# Autodesk Inventor assembly: Wechselmechnanik
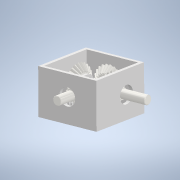
[picture p0: Inventor's stored thumbnail of the model, 180x180]
Saved by Autodesk Inventor 2021 (Build 250183000, 183)
## iProperties
Created: 2021-01-24
Part Number: Wechselmechnanik
Document SubType Name: Assembly
Designer: Jaro Machnow
Author: Jaro Machnow
## Documents named in this file (14)
- C:\Users\LETPJG\Documents\Inventor\zahnstange\Amphibienfahrzeug\Wechsel zwischen Land und Wasser\Mechanik_zum_Wechseln\Wechselmechnanik\Wechselmechnanik.iam
- C:\Users\LETPJG\Documents\Inventor\zahnstange\Amphibienfahrzeug\Wechsel zwischen Land und Wasser\Mechanik_zum_Wechseln\Wechselmechnanik\Konstruktions-Assistent\Kegelräder1.iam
- C:\Users\LETPJG\Documents\Inventor\zahnstange\Amphibienfahrzeug\Wechsel zwischen Land und Wasser\Mechanik_zum_Wechseln\Welle1.ipt
- C:\Users\LETPJG\Documents\Inventor\zahnstange\Amphibienfahrzeug\Wechsel zwischen Land und Wasser\Mechanik_zum_Wechseln\Welle2.ipt
- C:\Users\LETPJG\Documents\Inventor\zahnstange\Amphibienfahrzeug\Wechsel zwischen Land und Wasser\Mechanik_zum_Wechseln\Wechselmechnanik\Konstruktions-Assistent\Lager1.iam
- C:\Users\LETPJG\Documents\Inventor\zahnstange\Amphibienfahrzeug\Wechsel zwischen Land und Wasser\Mechanik_zum_Wechseln\Wechselmechnanik\Konstruktions-Assistent\Kegelräder3.iam
- C:\Users\LETPJG\Documents\Inventor\zahnstange\Amphibienfahrzeug\Wechsel zwischen Land und Wasser\Wechselmechanik\Klappmechanismus\Lager1.iam
- C:\Users\LETPJG\Documents\Inventor\zahnstange\Amphibienfahrzeug\Wechsel zwischen Land und Wasser\Mechanik_zum_Wechseln\Hülle.ipt
- C:\Users\LETPJG\Documents\Inventor\zahnstange\Amphibienfahrzeug\Wechsel zwischen Land und Wasser\Mechanik_zum_Wechseln\Schiebeteil.ipt
- C:\Users\LETPJG\Documents\Inventor\zahnstange\Amphibienfahrzeug\Wechsel zwischen Land und Wasser\Mechanik_zum_Wechseln\Abstandsring.ipt
- C:\Users\LETPJG\Documents\Inventor\zahnstange\Amphibienfahrzeug\Wechsel zwischen Land und Wasser\Mechanik_zum_Wechseln\Zahnstange.iam
- C:\Users\LETPJG\Documents\Inventor\zahnstange\Amphibienfahrzeug\Wechsel zwischen Land und Wasser\Mechanik_zum_Wechseln\Wechselmechnanik\Konstruktions-Assistent\Keilverbindung2.iam
- C:\Users\LETPJG\Documents\Inventor\zahnstange\Amphibienfahrzeug\Wechsel zwischen Land und Wasser\Mechanik_zum_Wechseln\Welle3.ipt
- C:\Users\LETPJG\Documents\Inventor\zahnstange\Amphibienfahrzeug\Wechsel zwischen Land und Wasser\Mechanik_zum_Wechseln\Wechselmechnanik\Konstruktions-Assistent\Keilverbindung3.iam
## Components (25 placed, 8 different names)
1. Kegelräder:1 [sub-assembly] — Passend:2, Passend:18, Passend:20
2. Welle:1 — Passend:4, Winkel:2, Passend:22, Passend:53, Fluchtend:3, Winkel:6, Passend:59, Passend:60
3. Welle:1 — Passend:2, Passend:6, Passend:7, Passend:12, Passend:16, Passend:19, Passend:31, Passend:45
4. Lager:1 [sub-assembly] — Passend:7, Passend:17, Passend:47
5. Kegelräder:2 [sub-assembly] — Passend:4, Winkel:2, Passend:24
6. Lager:2 [sub-assembly] — Passend:6, Passend:48
7. Hülle:1 — Passend:12, Passend:27, Passend:29, Passend:30, Passend:40, Passend:41, Passend:42, Passend:51, Passend:52, Passend:54, Passend:55, Passend:56, Fluchtend:4, Passend:60
8. Lager:3 [sub-assembly] — Passend:27, Passend:28, Passend:52, Passend:53
9. Schiebeteil:1 — Passend:45, Passend:46, Passend:47, Passend:48, Passend:49, Passend:50, Passend:51
10. Abstandsring:1 — Passend:16, Passend:17, Passend:18
11. Abstandsring:2 — Passend:19, Passend:20
12. Zahnstange:1 [sub-assembly] — Passend:54, Winkel:5
13. Keilverbindung:1 [sub-assembly] — Fluchtend:3, Winkel:6, Passend:59
14. Abstandsring:3 — Passend:22, Passend:24, Passend:28
15. Lager:4 [sub-assembly] — Passend:29, Passend:30, Passend:31
16. Kegelräder:3 [sub-assembly]
17. Welle:2 — Passend:40, Passend:43, Passend:46
18. Lager:5 [sub-assembly] — Passend:49
19. Lager:6 [sub-assembly] — Passend:50
20. Abstandsring:4
21. Abstandsring:5
22. Lager:7 [sub-assembly] — Passend:41, Passend:42, Passend:43
23. Lager:8 [sub-assembly] — Passend:55, Passend:56, Passend:57
24. Welle:1 — Passend:57, Fluchtend:2, Winkel:4, Passend:58, Winkel:5, Fluchtend:4
25. Keilverbindung:2 [sub-assembly] — Fluchtend:2, Winkel:4, Passend:58
## Relationships (52: Mate 45, Angle 4, Flush 3)
- Passend:2 [Mate]: Kegelräder:1 ↔ Welle:1
- Passend:4 [Mate]: Welle:1 ↔ Kegelräder:2
- Passend:6 [Mate]: Welle:1 ↔ Lager:2
- Passend:7 [Mate]: Welle:1 ↔ Lager:1
- Passend:12 [Mate]: Welle:1 ↔ Hülle:1
- Passend:16 [Mate]: Welle:1 ↔ Abstandsring:1
- Passend:17 [Mate]: Lager:1 ↔ Abstandsring:1
- Passend:18 [Mate]: Kegelräder:1 ↔ Abstandsring:1
- Passend:19 [Mate]: Welle:1 ↔ Abstandsring:2
- Passend:20 [Mate]: Kegelräder:1 ↔ Abstandsring:2
- Winkel:2 [Angle] (99.5917 deg): Welle:1 ↔ Kegelräder:2
- Passend:22 [Mate]: Welle:1 ↔ Abstandsring:3
- Passend:24 [Mate]: Kegelräder:2 ↔ Abstandsring:3
- Passend:27 [Mate]: Hülle:1 ↔ Lager:3
- Passend:28 [Mate]: Lager:3 ↔ Abstandsring:3
- Passend:29 [Mate]: Hülle:1 ↔ Lager:4
- Passend:30 [Mate]: Hülle:1 ↔ Lager:4
- Passend:31 [Mate]: Welle:1 ↔ Lager:4
- [Mate]: Kegelräder:3 ↔ Welle:2
- [Mate]: Welle:2 ↔ Lager:6
- [Mate]: Welle:2 ↔ Lager:5
- [Mate]: Welle:2 ↔ Abstandsring:4
- [Mate]: Lager:5 ↔ Abstandsring:4
- [Mate]: Kegelräder:3 ↔ Abstandsring:4
- [Mate]: Welle:2 ↔ Abstandsring:5
- [Mate]: Kegelräder:3 ↔ Abstandsring:5
- Passend:40 [Mate]: Hülle:1 ↔ Welle:2
- Passend:41 [Mate]: Hülle:1 ↔ Lager:7
- Passend:42 [Mate]: Hülle:1 ↔ Lager:7
- Passend:43 [Mate]: Welle:2 ↔ Lager:7
- Passend:45 [Mate]: Welle:1 ↔ Schiebeteil:1
- Passend:46 [Mate]: Schiebeteil:1 ↔ Welle:2
- Passend:47 [Mate]: Lager:1 ↔ Schiebeteil:1
- Passend:48 [Mate]: Lager:2 ↔ Schiebeteil:1
- Passend:49 [Mate]: Schiebeteil:1 ↔ Lager:5
- Passend:50 [Mate]: Schiebeteil:1 ↔ Lager:6
- Passend:51 [Mate]: Hülle:1 ↔ Schiebeteil:1
- Passend:52 [Mate]: Hülle:1 ↔ Lager:3
- Passend:53 [Mate]: Welle:1 ↔ Lager:3
- Passend:54 [Mate]: Hülle:1 ↔ Zahnstange:1
- Passend:55 [Mate]: Hülle:1 ↔ Lager:8
- Passend:56 [Mate]: Hülle:1 ↔ Lager:8
- Passend:57 [Mate]: Lager:8 ↔ Welle:1
- Fluchtend:2 [Flush] (0.9339 mm): Welle:1 ↔ Keilverbindung:2
- Winkel:4 [Angle] (0 deg): Welle:1 ↔ Keilverbindung:2
- Passend:58 [Mate]: Welle:1 ↔ Keilverbindung:2
- Winkel:5 [Angle] (66.0073 deg): Zahnstange:1 ↔ Welle:1
- Fluchtend:3 [Flush] (1.5781 mm): Welle:1 ↔ Keilverbindung:1
- Winkel:6 [Angle] (0 deg): Welle:1 ↔ Keilverbindung:1
- Passend:59 [Mate]: Welle:1 ↔ Keilverbindung:1
- Fluchtend:4 [Flush] (-1 mm): Hülle:1 ↔ Welle:1
- Passend:60 [Mate]: Welle:1 ↔ Hülle:1
## Named parameters: d46_d28 = 0 mm, d47_d29 = 0 mm, d48_d25 = 0 mm, d49_d26 = 0 mm, d50_d27 = 0 mm, d51_d1 = 0 mm, d52_d11 = 0 mm, d53_d12 = 0 mm
